# Autodesk Inventor assembly: frameAssembly
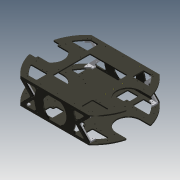
[picture p0: Inventor's stored thumbnail of the model, 180x180]
Saved by Autodesk Inventor 2018 (Build 220112000, 112)
## iProperties
Created: 2020-06-03
Part Number: frameAssembly
Document SubType Name: Assembly
Designer: anirudh
Author: anirudh
## Documents named in this file (5)
- D:\Silicon Sharks\2019-2020\prototype4\frameAssembly.iam
- D:\Silicon Sharks\2019-2020\prototype4\bottomPlate.ipt
- D:\Silicon Sharks\2019-2020\prototype4\topPlate.ipt
- D:\Silicon Sharks\2019-2020\prototype4\sidePlate.ipt
- D:\Silicon Sharks\2019-2020\prototype4\frameBracket.ipt
## Components (8 placed, 4 different names)
1. bottomPlate:1 — Mate:1, Mate:2, Mate:3, Mate:4, Mate:5, Mate:6, Mate:11, Mate:14, Mate:20
2. topPlate:1 — Mate:7, Mate:8, Mate:9, Mate:17
3. sidePlate:1 — Mate:4, Mate:5, Mate:6, Mate:7, Mate:8, Mate:9, Mate:10, Mate:12, Mate:13, Mate:15
4. sidePlate:2 — Mate:1, Mate:2, Mate:3, Mate:16, Mate:18, Mate:19, Mate:21
5. frameBracket:1 — Mate:13, Mate:14, Mate:15
6. frameBracket:2 — Mate:10, Mate:11, Mate:12
7. frameBracket:3 — Mate:16, Mate:17, Mate:18
8. frameBracket:4 — Mate:19, Mate:20, Mate:21
## Relationships (21: Mate 21)
- Mate:1: bottomPlate:1 ↔ sidePlate:2
- Mate:2: bottomPlate:1 ↔ sidePlate:2
- Mate:3: bottomPlate:1 ↔ sidePlate:2
- Mate:4: bottomPlate:1 ↔ sidePlate:1
- Mate:5: bottomPlate:1 ↔ sidePlate:1
- Mate:6: bottomPlate:1 ↔ sidePlate:1
- Mate:7: topPlate:1 ↔ sidePlate:1
- Mate:8: topPlate:1 ↔ sidePlate:1
- Mate:9: topPlate:1 ↔ sidePlate:1
- Mate:10: sidePlate:1 ↔ frameBracket:2
- Mate:11: bottomPlate:1 ↔ frameBracket:2
- Mate:12: sidePlate:1 ↔ frameBracket:2
- Mate:13: sidePlate:1 ↔ frameBracket:1
- Mate:14: bottomPlate:1 ↔ frameBracket:1
- Mate:15: sidePlate:1 ↔ frameBracket:1
- Mate:16: sidePlate:2 ↔ frameBracket:3
- Mate:17: topPlate:1 ↔ frameBracket:3
- Mate:18: sidePlate:2 ↔ frameBracket:3
- Mate:19: sidePlate:2 ↔ frameBracket:4
- Mate:20: bottomPlate:1 ↔ frameBracket:4
- Mate:21: sidePlate:2 ↔ frameBracket:4
